# Autodesk Inventor assembly: odometer_block
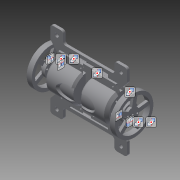
[picture p0: Inventor's stored thumbnail of the model, 180x180]
Saved by Autodesk Inventor 2015 (Build 190159000, 159)
## iProperties
Created: 2015-07-19
Part Number: odometer_block
Document SubType Name: Assembly
Designer: astralien3000
Author: astralien3000
## Documents named in this file (3)
- C:\Users\astralien3000\Desktop\ceres\meca\v2016\odometer_block.iam
- C:\Users\astralien3000\Desktop\ceres\meca\v2016\odometer_base.ipt
- C:\Users\astralien3000\Desktop\ceres\meca\v2016\encoder_block.iam
## Components (3 placed, 2 different names)
1. odometer_base:1 — Placage:1, Placage:2, Placage:3, Placage:4, Placage:5, Placage:6, Placage:7, Placage:8, Placage:9, Placage:10, Placage:11, Placage:12, Placage:13
2. encoder_block:1 [sub-assembly] — Placage:7, Placage:8, Placage:9, Placage:10, Placage:11
3. encoder_block:2 [sub-assembly] — Placage:4, Placage:5, Placage:6, Placage:12, Placage:13
## Relationships (13: Mate 13)
- Placage:1 [Mate]: odometer_base:1
- Placage:2 [Mate]: odometer_base:1
- Placage:3 [Mate]: odometer_base:1
- Placage:4 [Mate]: odometer_base:1 ↔ encoder_block:2
- Placage:5 [Mate]: odometer_base:1 ↔ encoder_block:2
- Placage:6 [Mate]: odometer_base:1 ↔ encoder_block:2
- Placage:7 [Mate]: odometer_base:1 ↔ encoder_block:1
- Placage:8 [Mate]: odometer_base:1 ↔ encoder_block:1
- Placage:9 [Mate]: odometer_base:1 ↔ encoder_block:1
- Placage:10 [Mate]: odometer_base:1 ↔ encoder_block:1
- Placage:11 [Mate]: odometer_base:1 ↔ encoder_block:1
- Placage:12 [Mate]: odometer_base:1 ↔ encoder_block:2
- Placage:13 [Mate]: odometer_base:1 ↔ encoder_block:2
